# Autodesk Inventor assembly: estação_bga_2
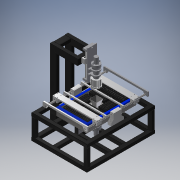
[picture p0: Inventor's stored thumbnail of the model, 180x180]
Saved by Autodesk Inventor 2018 (Build 220112000, 112)
## iProperties
Created: 2018-07-20
Part Number: estação_bga_2
Material: Genérico
Document SubType Name: Assembly
Designer: Usuario
Mass: 28977.3 g
Surface Area: 37496.8 cm^2
Volume: 6730.78 cm^3
Density: 4.30519 g/cm^3
Author: Usuario
## Documents named in this file (9)
- C:\Users\Usuario\Desktop\pecas_3d-20180530T120808Z-001\pecas_3d\estação_bga_2.iam
- C:\Users\Usuario\Desktop\pecas_3d-20180530T120808Z-001\pecas_3d\mesa_aquecimento_fresamento.iam
- C:\Users\Usuario\Desktop\pecas_3d-20180530T120808Z-001\pecas_3d\estrutura.iam
- C:\Users\Usuario\Desktop\pecas_3d-20180530T120808Z-001\pecas_3d\mesa_suporte_de_placa.iam
- C:\Users\Usuario\Desktop\pecas_3d-20180530T120808Z-001\pecas_3d\cabeça_superior.iam
- C:\Users\Usuario\Desktop\pecas_3d-20180530T120808Z-001\pecas_3d\cabeça_inferior.iam
- C:\Users\Usuario\Desktop\pecas_3d-20180530T120808Z-001\pecas_3d\ventilador_tangencial_referencia.ipt
- C:\Users\Usuario\Desktop\pecas_3d-20180530T120808Z-001\pecas_3d\bocal_inferior.ipt
- C:\Users\Usuario\Desktop\pecas_3d-20180530T120808Z-001\pecas_3d\ApoioBocalInferior_.ipt
## Components (8 placed, 8 different names)
1. mesa_aquecimento_fresamento:1 [sub-assembly] — Coincidência:11, Coincidência:14, Ângulo:1, Coincidência:15, Alinhamento:6, Coincidência:16
2. estrutura:1 [sub-assembly] — Coincidência:4, Coincidência:5, Coincidência:6, Alinhamento:2, Coincidência:8, Coincidência:14
3. mesa_suporte_de_placa:1 [sub-assembly] — Coincidência:15, Alinhamento:6, Coincidência:16
4. cabeça_inferior:1 [sub-assembly] — Coincidência:7, Alinhamento:3, Coincidência:9, Coincidência:10, Alinhamento:4, Alinhamento:5, Coincidência:11
5. cabeça_superior:2 [sub-assembly] — Coincidência:4, Coincidência:5, Alinhamento:5
6. ventilador_tangencial_referencia:1
7. bocal_inferior:1 — Coincidência:9, Coincidência:10
8. ApoioBocalInferior_:1 — Coincidência:6, Alinhamento:2, Coincidência:7, Alinhamento:3, Coincidência:8, Alinhamento:4, Ângulo:1
## Relationships (17: Mate 11, Flush 5, Angle 1)
- Coincidência:4 [Mate] (-45 mm): estrutura:1 ↔ cabeça_superior:2
- Coincidência:5 [Mate]: estrutura:1 ↔ cabeça_superior:2
- Coincidência:6 [Mate]: estrutura:1 ↔ ApoioBocalInferior_:1
- Alinhamento:2 [Flush]: estrutura:1 ↔ ApoioBocalInferior_:1
- Coincidência:7 [Mate]: cabeça_inferior:1 ↔ ApoioBocalInferior_:1
- Alinhamento:3 [Flush] (28 mm): cabeça_inferior:1 ↔ ApoioBocalInferior_:1
- Coincidência:8 [Mate]: estrutura:1 ↔ ApoioBocalInferior_:1
- Coincidência:9 [Mate]: cabeça_inferior:1 ↔ bocal_inferior:1
- Coincidência:10 [Mate]: cabeça_inferior:1 ↔ bocal_inferior:1
- Alinhamento:4 [Flush] (80 mm): cabeça_inferior:1 ↔ ApoioBocalInferior_:1
- Alinhamento:5 [Flush]: cabeça_inferior:1 ↔ cabeça_superior:2
- Coincidência:11 [Mate]: mesa_aquecimento_fresamento:1 ↔ cabeça_inferior:1
- Coincidência:14 [Mate]: mesa_aquecimento_fresamento:1 ↔ estrutura:1
- Ângulo:1 [Angle] (90 deg): mesa_aquecimento_fresamento:1 ↔ ApoioBocalInferior_:1
- Coincidência:15 [Mate] (17.016 mm): mesa_aquecimento_fresamento:1 ↔ mesa_suporte_de_placa:1
- Alinhamento:6 [Flush]: mesa_aquecimento_fresamento:1 ↔ mesa_suporte_de_placa:1
- Coincidência:16 [Mate] (40.48 mm): mesa_aquecimento_fresamento:1 ↔ mesa_suporte_de_placa:1
